# Autodesk Inventor assembly: am-3076a_DART_6_Extended
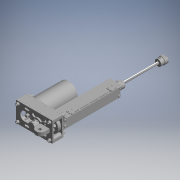
[picture p0: Inventor's stored thumbnail of the model, 180x180]
Saved by Autodesk Inventor 2017 SP1 (Build 210196100, 196)
## iProperties
Created: 2016-01-12
Part Number: am-3076a_DART_6_Extended
Description: STEP AP203
Document SubType Name: Assembly
Designer: steele
Sending System: SolidWorks 2014
Preprocessor: SwSTEP 2.0
Title: am-3076a DART 6.STEP
Revision Number: ANY
## Documents named in this file (5)
- D:\snobotics\CAD-MfgResources\Andy-Mark\Linear Actuators\DART 6 in Actuator AM-3076a\am-3076a_DART_6_Extended.iam
- D:\snobotics\CAD-MfgResources\Andy-Mark\Linear Actuators\DART 6 in Actuator AM-3076a\am-3275 DART Motor Module.iam
- D:\snobotics\CAD-MfgResources\Andy-Mark\Linear Actuators\DART 6 in Actuator AM-3076a\am-3289 DART 6 Lead Screw Module.iam
- D:\snobotics\CAD-MfgResources\Andy-Mark\Linear Actuators\DART 6 in Actuator AM-3076a\Dart Extension.ipt
- D:\snobotics\CAD-MfgResources\Andy-Mark\Linear Actuators\DART 6 in Actuator AM-3076a\am-3258 DART Ram Cap.ipt
## Components (4 placed, 4 different names)
1. am-3275 DART Motor Module_1 [sub-assembly]
2. am-3289 DART 6 Lead Screw Module_2 [sub-assembly] — Insert:1
3. Dart Extension:1 — Insert:1, Insert:2
4. am-3258 DART Ram Cap:1 — Insert:2
## Relationships (2: Insert 2)
- Insert:1: am-3289 DART 6 Lead Screw Module_2 ↔ Dart Extension:1
- Insert:2: Dart Extension:1 ↔ am-3258 DART Ram Cap:1
